# Autodesk Inventor assembly: WaferStack
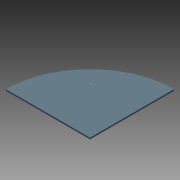
[picture p0: Inventor's stored thumbnail of the model, 180x180]
Saved by Autodesk Inventor 2011 SP1 (Build 150282100, 282)
## iProperties
Created: 2011-03-24
Part Number: WaferStack
Document SubType Name: Assembly
Designer: Andrew Zonenberg
Author: Andrew Zonenberg
## Documents named in this file (3)
- C:\Users\Andrew Zonenberg\Documents\programming\blackstart\mems\combdrive\WaferStack.iam
- C:\Users\Andrew Zonenberg\Documents\programming\blackstart\mems\combdrive\carrier-wafer.ipt
- C:\Users\Andrew Zonenberg\Documents\programming\blackstart\mems\combdrive\top-wafer.ipt
## Components (2 placed, 2 different names)
1. carrier-wafer:1 — Mate:1, Flush:1, Flush:2
2. top-wafer:1 — Mate:1, Flush:1, Flush:2
## Relationships (3: Flush 2, Mate 1)
- Mate:1: carrier-wafer:1 ↔ top-wafer:1
- Flush:1: carrier-wafer:1 ↔ top-wafer:1
- Flush:2: carrier-wafer:1 ↔ top-wafer:1
